# Autodesk Inventor assembly: Head
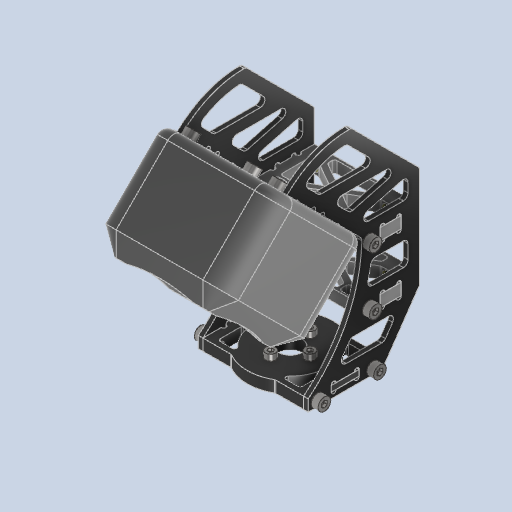
[picture p0: Inventor's stored thumbnail of the model, 512x512]
Saved by Autodesk Inventor 2022.5 (Build 265521000, 521)
## iProperties
Created: 2023-05-06
Part Number: Head
Document SubType Name: Assembly
Designer: Masato Kubotera
Author: Masato Kubotera
## Documents named in this file (8)
- C:\Users\Masato\Documents\Inventor\SUSTAINA-OP\ModelingFiles\UpperBody\Head\Head.iam
- C:\Users\Masato\Documents\Inventor\SUSTAINA-OP\ModelingFiles\UpperBody\Head\Head_neck_side_frame.ipt
- C:\Users\Masato\Documents\Inventor\SUSTAINA-OP\ModelingFiles\UpperBody\Head\Head_camera_unit.iam
- C:\Users\Masato\Documents\Inventor\SUSTAINA-OP\ModelingFiles\UpperBody\UpperBody_horn_frame.ipt
- C:\Users\Masato\Documents\Inventor\SUSTAINA-OP\ModelingFiles\COTS\Screw\UC-0306.ipt
- C:\Users\Masato\Documents\Inventor\SUSTAINA-OP\ModelingFiles\COTS\Screw\UC-2610.ipt
- C:\Users\Masato\Documents\Inventor\SUSTAINA-OP\ModelingFiles\COTS\Washer\TT-2532-20.ipt
- C:\Users\Masato\Documents\Inventor\SUSTAINA-OP\ModelingFiles\UpperBody\Head\Head_neck_diagonal.iam
## Components (19 placed, 7 different names)
1. Head_camera_unit:1 [sub-assembly] — Mate:1, Mate:2, メイト:3, メイト:4
2. Head_neck_diagonal:1 [sub-assembly] — 挿入:14, 角度:1, 角度:2
3. Head_neck_diagonal:2 [sub-assembly] — 挿入:15, 角度:3
4. UpperBody_horn_frame:1 — 挿入:1, 挿入:2, 挿入:3, 挿入:4, 挿入:9, 挿入:10, 挿入:11, 挿入:12, 挿入:13, メイト:5, メイト:6
5. Head_neck_side_frame:1 — Mate:1, メイト:3, メイト:4, フラッシュ:4, フラッシュ:5, 挿入:1, 挿入:2, 挿入:5, 挿入:6, 挿入:14, 挿入:15, 挿入:16, 挿入:17
6. Head_neck_side_frame:2 — Mate:2, フラッシュ:4, フラッシュ:5, 挿入:3, 挿入:4, 挿入:7, 挿入:8, 挿入:18, 挿入:19
7. TT-2532-20:1 — 挿入:13, メイト:7
8. UC-0306:1 — 挿入:5
9. UC-0306:2 — 挿入:6
10. UC-0306:3 — 挿入:7
11. UC-0306:4 — 挿入:8
12. UC-0306:5 — 挿入:16
13. UC-0306:6 — 挿入:17
14. UC-0306:7 — 挿入:18
15. UC-0306:8 — 挿入:19
16. UC-2610:1 — 挿入:9
17. UC-2610:2 — 挿入:10
18. UC-2610:3 — 挿入:12
19. UC-2610:4 — 挿入:11
## Relationships (31: Insert 19, Mate 7, Angle 3, Flush 2)
- Mate:1: Head_camera_unit:1 ↔ Head_neck_side_frame:1
- Mate:2: Head_camera_unit:1 ↔ Head_neck_side_frame:2
- メイト:3 [Mate] (0.05 mm): Head_camera_unit:1 ↔ Head_neck_side_frame:1
- メイト:4 [Mate] (0.05 mm): Head_camera_unit:1 ↔ Head_neck_side_frame:1
- フラッシュ:4 [Flush]: Head_neck_side_frame:1 ↔ Head_neck_side_frame:2
- フラッシュ:5 [Flush]: Head_neck_side_frame:1 ↔ Head_neck_side_frame:2
- 挿入:1 [Insert]: UpperBody_horn_frame:1 ↔ Head_neck_side_frame:1
- 挿入:2 [Insert]: UpperBody_horn_frame:1 ↔ Head_neck_side_frame:1
- 挿入:3 [Insert]: UpperBody_horn_frame:1 ↔ Head_neck_side_frame:2
- 挿入:4 [Insert]: UpperBody_horn_frame:1 ↔ Head_neck_side_frame:2
- 挿入:5 [Insert]: Head_neck_side_frame:1 ↔ UC-0306:1
- 挿入:6 [Insert]: Head_neck_side_frame:1 ↔ UC-0306:2
- 挿入:7 [Insert]: Head_neck_side_frame:2 ↔ UC-0306:3
- 挿入:8 [Insert]: Head_neck_side_frame:2 ↔ UC-0306:4
- 挿入:9 [Insert]: UpperBody_horn_frame:1 ↔ UC-2610:1
- 挿入:10 [Insert]: UpperBody_horn_frame:1 ↔ UC-2610:2
- 挿入:11 [Insert]: UpperBody_horn_frame:1 ↔ UC-2610:4
- 挿入:12 [Insert]: UpperBody_horn_frame:1 ↔ UC-2610:3
- 挿入:13 [Insert]: UpperBody_horn_frame:1 ↔ TT-2532-20:1
- 挿入:14 [Insert]: Head_neck_diagonal:1 ↔ Head_neck_side_frame:1
- 挿入:15 [Insert]: Head_neck_diagonal:2 ↔ Head_neck_side_frame:1
- 挿入:16 [Insert]: Head_neck_side_frame:1 ↔ UC-0306:5
- 挿入:17 [Insert]: Head_neck_side_frame:1 ↔ UC-0306:6
- 挿入:18 [Insert]: Head_neck_side_frame:2 ↔ UC-0306:7
- 挿入:19 [Insert]: Head_neck_side_frame:2 ↔ UC-0306:8
- 角度:1 [Angle] (0 deg): Head_neck_diagonal:1
- 角度:2 [Angle] (0 deg): Head_neck_diagonal:1
- 角度:3 [Angle] (0 deg): Head_neck_diagonal:2
- メイト:5 [Mate]: UpperBody_horn_frame:1
- メイト:6 [Mate]: UpperBody_horn_frame:1
- メイト:7 [Mate]: TT-2532-20:1
